# Autodesk Inventor assembly: ChassisFrame
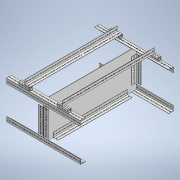
[picture p0: Inventor's stored thumbnail of the model, 180x180]
Saved by Autodesk Inventor 2020 (Build 240168000, 168)
## iProperties
Created: 2021-11-11
Part Number: ChassisFrame
Document SubType Name: Assembly
Designer: 17185
Author: 17185
## Documents named in this file (6)
- C:\Users\17185\Desktop\chassis draft\Chassis Frame\ChassisFrame.iam
- C:\Users\17185\Desktop\chassis draft\Chassis Frame\ChassisWall.ipt
- C:\Users\17185\Desktop\chassis draft\Chassis Frame\AngleBar - 8 in.ipt
- C:\Users\17185\Desktop\chassis draft\Chassis Frame\AngleBar - 2 ft.ipt
- C:\Users\17185\Desktop\chassis draft\Chassis Frame\SquareTube.ipt
- C:\Users\17185\Desktop\chassis draft\Chassis Frame\AngleBar - 2.5 ft.ipt
## Components (17 placed, 5 different names)
1. AngleBar - 8 in:3 — Flush:10, Flush:13, Mate:26, Flush:19
2. AngleBar - 8 in:4 — Flush:10, Flush:13, Mate:22, Flush:18
3. AngleBar - 2 ft:1 — Flush:18, Mate:27, Mate:28, Flush:23, Flush:24, Flush:27, Flush:28
4. AngleBar - 2 ft:2 — Mate:29, Mate:30, Flush:21, Flush:22
5. AngleBar - 2 ft:3 — Flush:20
6. AngleBar - 2 ft:4 — Mate:24, Mate:25
7. AngleBar - 8 in:5 — Flush:11, Mate:20, Flush:17
8. AngleBar - 8 in:6 — Flush:11, Mate:21, Flush:17, Flush:19
9. ChassisWall:1 — Mate:20, Mate:21, Mate:22, Mate:23, Mate:24, Mate:25, Mate:26
10. AngleBar - 2 ft:1 — Flush:14, Flush:15, Flush:20
11. AngleBar - 2 ft:2 — Mate:23, Flush:14, Flush:15
12. SquareTube:1 — Mate:27, Flush:24, Flush:25, Flush:27, Mate:35
13. SquareTube:2 — Mate:29, Flush:22, Flush:26
14. SquareTube:3 — Mate:30, Flush:21, Flush:25
15. SquareTube:4 — Mate:28, Flush:23, Flush:26, Flush:28
16. AngleBar - 2.5 ft:1
17. AngleBar - 2.5 ft:2 — Mate:35
## Relationships (29: Flush 17, Mate 12)
- Flush:10: AngleBar - 8 in:3 ↔ AngleBar - 8 in:4
- Flush:11: AngleBar - 8 in:5 ↔ AngleBar - 8 in:6
- Flush:13: AngleBar - 8 in:3 ↔ AngleBar - 8 in:4
- Mate:20: AngleBar - 8 in:5 ↔ ChassisWall:1
- Mate:21: AngleBar - 8 in:6 ↔ ChassisWall:1
- Mate:22: AngleBar - 8 in:4 ↔ ChassisWall:1
- Mate:23: ChassisWall:1 ↔ AngleBar - 2 ft:2
- Flush:14: AngleBar - 2 ft:1 ↔ AngleBar - 2 ft:2
- Flush:15: AngleBar - 2 ft:1 ↔ AngleBar - 2 ft:2
- Mate:24: AngleBar - 2 ft:4 ↔ ChassisWall:1
- Mate:25: AngleBar - 2 ft:4 ↔ ChassisWall:1
- Flush:17: AngleBar - 8 in:5 ↔ AngleBar - 8 in:6
- Flush:18: AngleBar - 8 in:4 ↔ AngleBar - 2 ft:1
- Mate:26: AngleBar - 8 in:3 ↔ ChassisWall:1
- Flush:19: AngleBar - 8 in:3 ↔ AngleBar - 8 in:6
- Flush:20: AngleBar - 2 ft:3 ↔ AngleBar - 2 ft:1
- Mate:27: AngleBar - 2 ft:1 ↔ SquareTube:1
- Mate:28: AngleBar - 2 ft:1 ↔ SquareTube:4
- Mate:29: AngleBar - 2 ft:2 ↔ SquareTube:2
- Mate:30: AngleBar - 2 ft:2 ↔ SquareTube:3
- Flush:21: AngleBar - 2 ft:2 ↔ SquareTube:3
- Flush:22: AngleBar - 2 ft:2 ↔ SquareTube:2
- Flush:23: AngleBar - 2 ft:1 ↔ SquareTube:4
- Flush:24: AngleBar - 2 ft:1 ↔ SquareTube:1
- Flush:25: SquareTube:1 ↔ SquareTube:3
- Flush:26: SquareTube:2 ↔ SquareTube:4
- Flush:27 (-101.6 mm): AngleBar - 2 ft:1 ↔ SquareTube:1
- Flush:28 (101.6 mm): AngleBar - 2 ft:1 ↔ SquareTube:4
- Mate:35: SquareTube:1 ↔ AngleBar - 2.5 ft:2
